# Autodesk Inventor assembly: Gear HS 60 tooth (free)
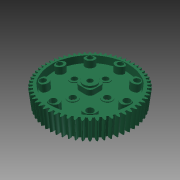
[picture p0: Inventor's stored thumbnail of the model, 180x180]
Saved by Autodesk Inventor 2015 (Build 190159000, 159)
## iProperties
Created: 2014-05-24
Part Number: Gear HS 60 tooth (free)
Document SubType Name: Assembly
Designer: Christopher
Author: Christopher
## Documents named in this file (3)
- C:\Users\Christopher\Documents\Inventor\VEX CAD Library\Motion\Gear HS 60 tooth (free).iam
- C:\Users\Christopher\Documents\Inventor\VEX CAD Library\Motion\Gear HS 60 tooth.ipt
- C:\Users\Christopher\Documents\Inventor\VEX CAD Library\Motion\Insert HS Plastic.ipt
## Components (3 placed, 2 different names)
1. Gear HS 60 tooth:1 — Mate:1, Mate:2, Angle:1, Angle:2, Mate:3, Mate:4
2. Insert HS Plastic:1 — Mate:2, Angle:1, Mate:4
3. Insert HS Plastic:2 — Mate:1, Angle:2, Mate:3
## Relationships (6: Mate 4, Angle 2)
- Mate:1: Gear HS 60 tooth:1 ↔ Insert HS Plastic:2
- Mate:2: Gear HS 60 tooth:1 ↔ Insert HS Plastic:1
- Angle:1 (0 deg): Gear HS 60 tooth:1 ↔ Insert HS Plastic:1
- Angle:2 (0 deg): Gear HS 60 tooth:1 ↔ Insert HS Plastic:2
- Mate:3: Gear HS 60 tooth:1 ↔ Insert HS Plastic:2
- Mate:4: Gear HS 60 tooth:1 ↔ Insert HS Plastic:1
